# Autodesk Inventor assembly: Projekat oktobar
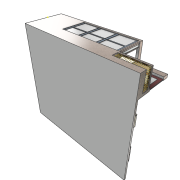
[picture p0: Inventor's stored thumbnail of the model, 180x180]
Saved by Autodesk Inventor 2020.2 (Build 242310000, 310)
## iProperties
Created: 2020-10-18
Part Number: Projekat oktobar
Document SubType Name: Assembly
Designer: User
Author: User
## Documents named in this file (9)
- D:\_Mihajlo Danilovic 358_19\Projekat oktobar.iam
- D:\_Mihajlo Danilovic 358_19\Projekat.ipt
- D:\_Mihajlo Danilovic 358_19\Radni sto.ipt
- D:\_Mihajlo Danilovic 358_19\Kauc.ipt
- D:\_Mihajlo Danilovic 358_19\Fotelja.ipt
- D:\_Mihajlo Danilovic 358_19\Sto u dnevnoj sobi.ipt
- D:\_Mihajlo Danilovic 358_19\Lampa.ipt
- D:\_Mihajlo Danilovic 358_19\Tepih.ipt
- D:\_Mihajlo Danilovic 358_19\Stolica.ipt
## Components (10 placed, 8 different names)
1. Projekat:1 — Mate:1, Mate:2, Mate:3, Mate:4, Mate:5, Mate:6, Mate:8, Mate:9, Mate:14, Mate:15, Mate:16, Mate:17, Mate:18, Mate:19
2. Radni sto:1 — Mate:1, Mate:2
3. Kauc:1 — Mate:3, Mate:4, Mate:7
4. Fotelja:1 — Mate:5
5. Sto u dnevnoj sobi:1 — Mate:6, Mate:7
6. Lampa:1 — Mate:8
7. Tepih:1 — Mate:9
8. Fotelja:2 — Mate:14
9. Fotelja:3 — Mate:15, Mate:18, Mate:19
10. Stolica:1 — Mate:16, Mate:17
## Relationships (15: Mate 15)
- Mate:1: Projekat:1 ↔ Radni sto:1
- Mate:2 (3500 mm): Projekat:1 ↔ Radni sto:1
- Mate:3: Projekat:1 ↔ Kauc:1
- Mate:4 (1500 mm): Projekat:1 ↔ Kauc:1
- Mate:5: Projekat:1 ↔ Fotelja:1
- Mate:6: Projekat:1 ↔ Sto u dnevnoj sobi:1
- Mate:7 (500 mm): Kauc:1 ↔ Sto u dnevnoj sobi:1
- Mate:8: Projekat:1 ↔ Lampa:1
- Mate:9: Projekat:1 ↔ Tepih:1
- Mate:14: Projekat:1 ↔ Fotelja:2
- Mate:15: Projekat:1 ↔ Fotelja:3
- Mate:16 (-15.392 mm): Projekat:1 ↔ Stolica:1
- Mate:17: Projekat:1 ↔ Stolica:1
- Mate:18: Projekat:1 ↔ Fotelja:3
- Mate:19 (20 mm): Projekat:1 ↔ Fotelja:3
